# Autodesk Inventor assembly: damascusCoverAssembly
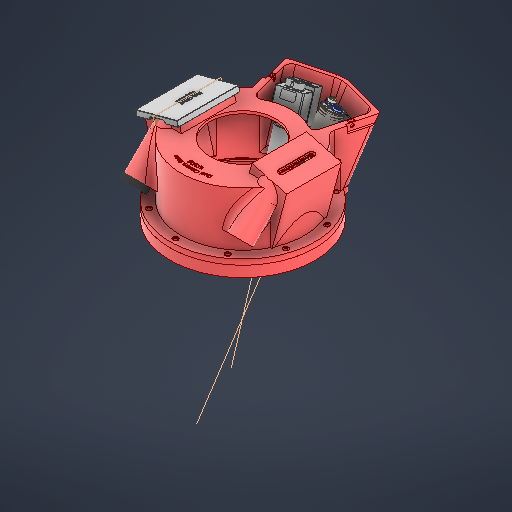
[picture p0: Inventor's stored thumbnail of the model, 512x512]
Saved by Autodesk Inventor 2026.2 (Build 302298000, 298)
## iProperties
Created: 2026-05-01
Part Number: damascusCoverAssembly
Document SubType Name: Assembly
Designer: mayhe
Author: mayhe
## Documents named in this file (13)
- C:\Users\mayhe\OneDrive\Documents\GitHub\In-situ-monitoring-of-powder-bed-fusion-additive-manufacturing\system_development\Damascus\V0.5\hardware development\damascusCoverAssembly.iam
- C:\Users\mayhe\OneDrive\Documents\GitHub\In-situ-monitoring-of-powder-bed-fusion-additive-manufacturing\system_development\Damascus\V0.5\hardware development\Parts\12mm Cover.ipt
- C:\Users\mayhe\OneDrive\Documents\GitHub\In-situ-monitoring-of-powder-bed-fusion-additive-manufacturing\system_development\Damascus\V0.5\hardware development\Parts\Build Plate with 35mm FOV Sketch.ipt
- C:\Users\mayhe\OneDrive\Documents\GitHub\In-situ-monitoring-of-powder-bed-fusion-additive-manufacturing\system_development\Damascus\V0.5\hardware development\Parts\sealRing.ipt
- C:\Users\mayhe\OneDrive\Documents\GitHub\In-situ-monitoring-of-powder-bed-fusion-additive-manufacturing\system_development\Damascus\V0.5\hardware development\Parts\Xi-410-Camera-with-29°-x-18°-Lens\Xi 410 Camera with 29° x.iam
- C:\Users\mayhe\OneDrive\Documents\GitHub\In-situ-monitoring-of-powder-bed-fusion-additive-manufacturing\system_development\Damascus\V0.5\hardware development\Parts\Optical Camera\Camera with 35mm.iam
- C:\Users\mayhe\OneDrive\Documents\GitHub\In-situ-monitoring-of-powder-bed-fusion-additive-manufacturing\system_development\Damascus\V0.5\hardware development\Parts\Antireflective Glass.ipt
- C:\Users\mayhe\OneDrive\Documents\GitHub\In-situ-monitoring-of-powder-bed-fusion-additive-manufacturing\system_development\Damascus\V0.5\hardware development\Parts\adapter-optical.ipt
- C:\Users\mayhe\OneDrive\Documents\GitHub\In-situ-monitoring-of-powder-bed-fusion-additive-manufacturing\system_development\Damascus\V0.5\hardware development\Parts\Event Camera\Triton2_asm.iam
- C:\Users\mayhe\OneDrive\Documents\GitHub\In-situ-monitoring-of-powder-bed-fusion-additive-manufacturing\system_development\Damascus\V0.5\hardware development\Parts\adapter-event.ipt
- C:\Users\mayhe\OneDrive\Documents\GitHub\In-situ-monitoring-of-powder-bed-fusion-additive-manufacturing\system_development\Damascus\V0.5\hardware development\Parts\Dual Camera Base.ipt
- C:\Users\mayhe\OneDrive\Documents\GitHub\In-situ-monitoring-of-powder-bed-fusion-additive-manufacturing\system_development\Damascus\V0.5\hardware development\Parts\Bolt Slot Covers.ipt
- C:\Users\mayhe\OneDrive\Documents\GitHub\In-situ-monitoring-of-powder-bed-fusion-additive-manufacturing\system_development\Damascus\V0.5\hardware development\Parts\WirePlugs.ipt
## Components (12 placed, 12 different names)
1. 12mm Cover:1 — Rotational:1, Rotational:2
2. Build Plate with 35mm FOV Sketch:1 — Rotational:1
3. sealRing:1 — Rotational:2, Rotational:5, Rotational:20
4. Xi 410 Camera with 29° x:1 [sub-assembly]
5. Antireflective Glass:1 — Rotational:5
6. Camera with 35mm:1 [sub-assembly] — Rotational:17
7. adapter-optical:1 — Rotational:17
8. Triton2_asm:1 [sub-assembly] — Rotational:19
9. adapter-event:1 — Rotational:19
10. Dual Camera Base:1 — Rotational:20, Mate:3, Mate:4, Mate:5, Rotational:21
11. Bolt Slot Covers:1 — Mate:3, Mate:4, Mate:5
12. WirePlugs:1 — Rotational:21
## Relationships (10: RevoluteJoint 7, Mate 3)
- Rotational:1 [RevoluteJoint] (-150 mm): 12mm Cover:1 ↔ Build Plate with 35mm FOV Sketch:1
- Rotational:2 [RevoluteJoint]: 12mm Cover:1 ↔ sealRing:1
- Rotational:5 [RevoluteJoint]: sealRing:1 ↔ Antireflective Glass:1
- Rotational:17 [RevoluteJoint]: Camera with 35mm:1 ↔ adapter-optical:1
- Rotational:19 [RevoluteJoint]: Triton2_asm:1 ↔ adapter-event:1
- Rotational:20 [RevoluteJoint]: sealRing:1 ↔ Dual Camera Base:1
- Mate:3: Dual Camera Base:1 ↔ Bolt Slot Covers:1
- Mate:4 (1.5 mm): Dual Camera Base:1 ↔ Bolt Slot Covers:1
- Mate:5 (1.5 mm): Dual Camera Base:1 ↔ Bolt Slot Covers:1
- Rotational:21 [RevoluteJoint]: Dual Camera Base:1 ↔ WirePlugs:1
